# Autodesk Inventor assembly: bundsamling
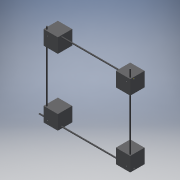
[picture p0: Inventor's stored thumbnail of the model, 180x180]
Saved by Autodesk Inventor 2018 (Build 220112000, 112)
## iProperties
Created: 2018-01-29
Part Number: bundsamling
Document SubType Name: Assembly
Designer: MikkelS
Author: MikkelS
## Documents named in this file (4)
- C:\Users\MikkelS\Documents\Inventor\Teknikproj2\bundsamling.iam
- C:\Users\MikkelS\Documents\Inventor\Teknikproj2\Bundhjørne1.ipt
- C:\Users\MikkelS\Documents\Inventor\Teknikproj2\gevindstang.ipt
- C:\Users\MikkelS\Documents\Inventor\Teknikproj2\Bundhjørnemirror.ipt
## Components (8 placed, 3 different names)
1. Bundhjørne1:1 — Flush:1, Flush:2, Flush:3, Mate:2, Mate:3, Flush:6
2. gevindstang:2 — Mate:2, Mate:4
3. gevindstang:3 — Mate:3, Mate:7
4. gevindstang:4 — Mate:5, Mate:6, Mate:10
5. Bundhjørnemirror:1 — Mate:4, Mate:5, Flush:6, Flush:7
6. Bundhjørne1:2 — Mate:6, Flush:7, Flush:9, Mate:8, Mate:10
7. Bundhjørnemirror:2 — Mate:7, Flush:9, Mate:9
8. gevindstang:5 — Mate:8, Mate:9
## Relationships (15: Mate 9, Flush 6)
- Flush:1: Bundhjørne1:1
- Flush:2: Bundhjørne1:1
- Flush:3: Bundhjørne1:1
- Mate:2: Bundhjørne1:1 ↔ gevindstang:2
- Mate:3: Bundhjørne1:1 ↔ gevindstang:3
- Mate:4: gevindstang:2 ↔ Bundhjørnemirror:1
- Mate:5: gevindstang:4 ↔ Bundhjørnemirror:1
- Mate:6: gevindstang:4 ↔ Bundhjørne1:2
- Flush:6: Bundhjørne1:1 ↔ Bundhjørnemirror:1
- Flush:7: Bundhjørnemirror:1 ↔ Bundhjørne1:2
- Mate:7: gevindstang:3 ↔ Bundhjørnemirror:2
- Flush:9: Bundhjørne1:2 ↔ Bundhjørnemirror:2
- Mate:8: Bundhjørne1:2 ↔ gevindstang:5
- Mate:9: Bundhjørnemirror:2 ↔ gevindstang:5
- Mate:10: gevindstang:4 ↔ Bundhjørne1:2
